# Autodesk Inventor assembly: ball-assembly
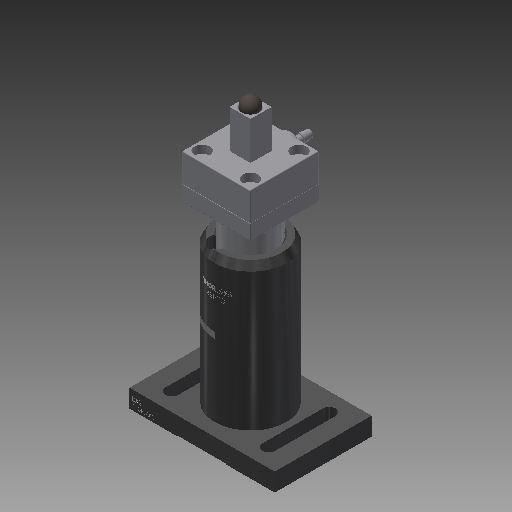
[picture p0: Inventor's stored thumbnail of the model, 512x512]
Saved by Autodesk Inventor 2019 (Build 230136000, 136)
## iProperties
Created: 2019-03-11
Part Number: ball-assembly
Document SubType Name: Assembly
Designer: Wilson Lab
Author: Wilson Lab
## Documents named in this file (7)
- C:\code\auditory-behavior-experiments\design-files\ball-assembly\ball-assembly.iam
- C:\code\auditory-behavior-experiments\design-files\ball-assembly\9mm_ball.ipt
- C:\code\auditory-behavior-experiments\design-files\ball-holder\9mm_ball_holder.ipt
- C:\code\auditory-behavior-experiments\design-files\vr-opto-assembly\RS3-Solidworks.ipt
- C:\code\auditory-behavior-experiments\design-files\vr-opto-assembly\RSHT3-Solidworks.ipt
- C:\code\auditory-behavior-experiments\design-files\ball-assembly\ball-holder-to-post-adapter.ipt
- C:\code\auditory-behavior-experiments\design-files\ball-assembly\BA2-Solidworks.ipt
## Components (6 placed, 6 different names)
1. 9mm_ball:1 — Rigid:2
2. 9mm_ball_holder:1 — Rigid:2, Rigid:5
3. RS3-Solidworks:1 — Rotational:1, Rigid:4
4. RSHT3-Solidworks:1 — Rotational:1, Rigid:6
5. ball-holder-to-post-adapter:1 — Rigid:4, Rigid:5
6. BA2-Solidworks:1 — Rigid:6
## Relationships (5: WeldJoint 4, RevoluteJoint 1)
- Rigid:2 [WeldJoint] (5.3 mm): 9mm_ball:1 ↔ 9mm_ball_holder:1
- Rotational:1 [RevoluteJoint] (10 mm): RS3-Solidworks:1 ↔ RSHT3-Solidworks:1
- Rigid:4 [WeldJoint]: RS3-Solidworks:1 ↔ ball-holder-to-post-adapter:1
- Rigid:5 [WeldJoint]: 9mm_ball_holder:1 ↔ ball-holder-to-post-adapter:1
- Rigid:6 [WeldJoint]: RSHT3-Solidworks:1 ↔ BA2-Solidworks:1
